# Autodesk Inventor assembly: Assembly1
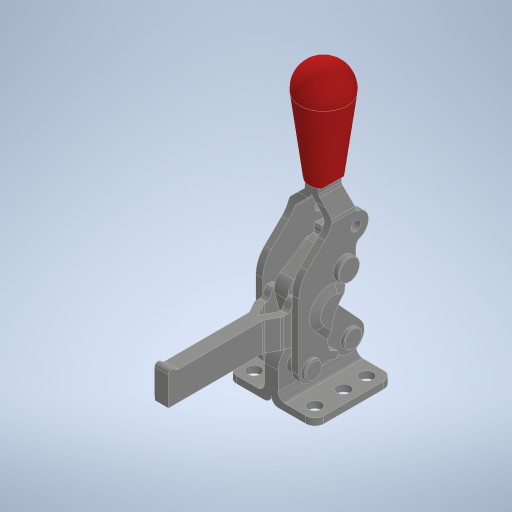
[picture p0: Inventor's stored thumbnail of the model, 512x512]
Saved by Autodesk Inventor 2024 (Build 280153000, 153)
## iProperties
Created: 2023-10-03
Part Number: Assembly1
Document SubType Name: Assembly
Designer: Shweta Raut
Mass: 36.7416 g
Surface Area: 210.515 cm^2
Volume: 36.7416 cm^3
Density: 1 g/cm^3
Author: Shweta Raut
## Documents named in this file (5)
- C:\Users\Shweta Raut\Documents\Assembly\Assembly1.iam
- C:\Users\Shweta Raut\Downloads\Assignment+Assembly+-+01_Question\Clamp_BASE.ipt
- C:\Users\Shweta Raut\Downloads\Assignment+Assembly+-+01_Question\Clamp_ARM.ipt
- C:\Users\Shweta Raut\Downloads\Assignment+Assembly+-+01_Question\Clamp_LINK.ipt
- C:\Users\Shweta Raut\Downloads\Assignment+Assembly+-+01_Question\Clamp_HANDLE.ipt
## Components (4 placed, 4 different names)
1. Clamp_BASE:1 — Mate:1, Flush:1, Mate:3, Flush:5, Angle:1
2. Clamp_ARM:1 — Mate:1, Flush:1, Mate:2, Flush:2, Flush:3, Flush:4
3. Clamp_LINK:1 — Mate:2, Flush:2, Flush:3, Flush:4, Mate:4
4. Clamp_HANDLE:1 — Mate:3, Flush:5, Mate:4, Angle:1
## Relationships (10: Flush 5, Mate 4, Angle 1)
- Mate:1: Clamp_BASE:1 ↔ Clamp_ARM:1
- Flush:1: Clamp_BASE:1 ↔ Clamp_ARM:1
- Mate:2: Clamp_ARM:1 ↔ Clamp_LINK:1
- Flush:2: Clamp_ARM:1 ↔ Clamp_LINK:1
- Flush:3: Clamp_ARM:1 ↔ Clamp_LINK:1
- Flush:4: Clamp_ARM:1 ↔ Clamp_LINK:1
- Mate:3: Clamp_BASE:1 ↔ Clamp_HANDLE:1
- Flush:5: Clamp_BASE:1 ↔ Clamp_HANDLE:1
- Mate:4: Clamp_LINK:1 ↔ Clamp_HANDLE:1
- Angle:1 (0 deg): Clamp_BASE:1 ↔ Clamp_HANDLE:1
